# Autodesk Inventor assembly: Assemlby_lightsheet_generator_passive_v2
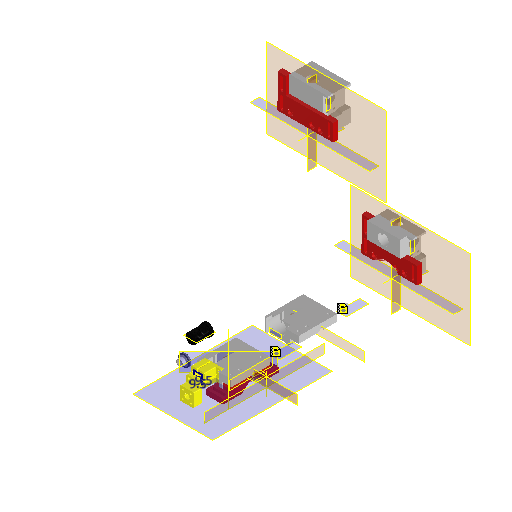
[picture p0: Inventor's stored thumbnail of the model, 512x512]
Saved by Autodesk Inventor 2025.3 (Build 293356000, 356)
## iProperties
Created: 2022-12-16
Part Number: Assemlby_lightsheet_generator_passive_v2
Document SubType Name: Assembly
Designer: UC2
Author: UC2
## Documents named in this file (11)
- C:\Users\benir\Documents\HoLiSheet\INVENTOR\Assemlby_lightsheet_generator_passive_v2.iam
- C:\Users\benir\Documents\HoLiSheet\INVENTOR\00_CCTV_lens_M12_25mm_5mp.ipt
- C:\Users\benir\Documents\HoLiSheet\INVENTOR\00_Thorlabs_LJ1878L1-A-Step.ipt
- C:\Users\benir\Documents\HoLiSheet\INVENTOR\00_SMAConnector_fiber copy.ipt
- C:\Users\benir\Documents\HoLiSheet\INVENTOR\30_Lightsheet_generator_passive_base_v1.ipt
- C:\Users\benir\Documents\HoLiSheet\INVENTOR\30_Lightsheet_generator_passive_lid_v1.ipt
- C:\Users\benir\Documents\HoLiSheet\INVENTOR\30_Laser_to_M12Adapter.ipt
- C:\Users\benir\Documents\HoLiSheet\INVENTOR\30_Laser_to_M12Adapter_9,5mm.ipt
- C:\Users\benir\Documents\HoLiSheet\INVENTOR\30_Lightsheet_generator_singlegalvo.ipt
- C:\Users\benir\Documents\HoLiSheet\INVENTOR\30_Lightsheet_generator_singlegalvo_1.ipt
- C:\Users\benir\Documents\HoLiSheet\INVENTOR\30_Lightsheet_generator_passive_lid_v1_singlegalvo.ipt
## Components (12 placed, 10 different names)
1. 30_Lightsheet_generator_passive_lid_v1:1 — Flush:7, Flush:8, Mate:1, Flush:9, Flush:10, Mate:4, Insert:2, Insert:3, Flush:12
2. 00_Thorlabs_LJ1878L1-A-Step:1 — Flush:7, Flush:8, Flush:9, Flush:10
3. 30_Lightsheet_generator_passive_base_v1:1 — Insert:2, Insert:3, Flush:12, Angle:2, Mate:7, Flush:13
4. 30_Laser_to_M12Adapter:1 — Angle:2, Mate:7, Flush:13
5. 00_CCTV_lens_M12_25mm_5mp:1
6. 00_SMAConnector_fiber copy:1
7. 30_Laser_to_M12Adapter_9,5mm:1
8. 30_Lightsheet_generator_passive_base_v1:2
9. 30_Lightsheet_generator_singlegalvo:1 — Insert:4, Angle:3
10. 30_Lightsheet_generator_passive_lid_v1:2 — Insert:4, Angle:3
11. 30_Lightsheet_generator_singlegalvo_1:1 — Insert:5, Insert:6
12. 30_Lightsheet_generator_passive_lid_v1_singlegalvo:1 — Insert:5, Insert:6
## Relationships (19: Flush 6, Mate 5, Insert 5, Angle 3)
- Flush:7 (1 mm): 30_Lightsheet_generator_passive_lid_v1:1 ↔ 00_Thorlabs_LJ1878L1-A-Step:1
- Flush:8: 30_Lightsheet_generator_passive_lid_v1:1 ↔ 00_Thorlabs_LJ1878L1-A-Step:1
- Mate:1: 30_Lightsheet_generator_passive_lid_v1:1
- Flush:9: 30_Lightsheet_generator_passive_lid_v1:1 ↔ 00_Thorlabs_LJ1878L1-A-Step:1
- Flush:10: 30_Lightsheet_generator_passive_lid_v1:1 ↔ 00_Thorlabs_LJ1878L1-A-Step:1
- Mate:4: 30_Lightsheet_generator_passive_lid_v1:1
- Mate:5
- Mate:6
- Angle:1 (90 deg)
- Insert:2: 30_Lightsheet_generator_passive_lid_v1:1 ↔ 30_Lightsheet_generator_passive_base_v1:1
- Insert:3: 30_Lightsheet_generator_passive_lid_v1:1 ↔ 30_Lightsheet_generator_passive_base_v1:1
- Flush:12: 30_Lightsheet_generator_passive_lid_v1:1 ↔ 30_Lightsheet_generator_passive_base_v1:1
- Angle:2 (270 deg): 30_Lightsheet_generator_passive_base_v1:1 ↔ 30_Laser_to_M12Adapter:1
- Mate:7: 30_Lightsheet_generator_passive_base_v1:1 ↔ 30_Laser_to_M12Adapter:1
- Flush:13 (3.5 mm): 30_Lightsheet_generator_passive_base_v1:1 ↔ 30_Laser_to_M12Adapter:1
- Insert:4: 30_Lightsheet_generator_singlegalvo:1 ↔ 30_Lightsheet_generator_passive_lid_v1:2
- Angle:3 (-90 deg): 30_Lightsheet_generator_singlegalvo:1 ↔ 30_Lightsheet_generator_passive_lid_v1:2
- Insert:5: 30_Lightsheet_generator_singlegalvo_1:1 ↔ 30_Lightsheet_generator_passive_lid_v1_singlegalvo:1
- Insert:6: 30_Lightsheet_generator_singlegalvo_1:1 ↔ 30_Lightsheet_generator_passive_lid_v1_singlegalvo:1
